# Autodesk Inventor assembly: Kolo+Opona
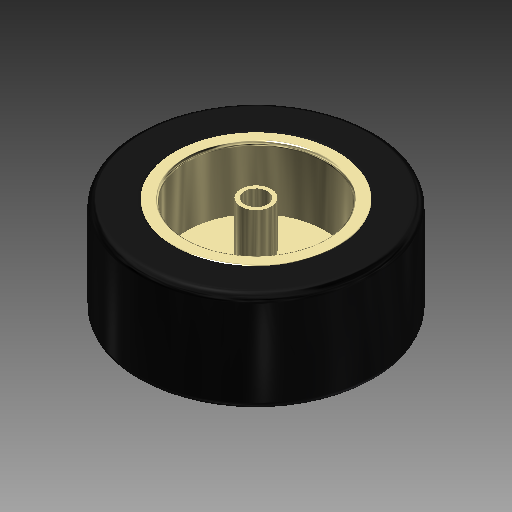
[picture p0: Inventor's stored thumbnail of the model, 512x512]
Saved by Autodesk Inventor 2017 (Build 210142000, 142)
## iProperties
Created: 2016-11-09
Part Number: Kolo+Opona
Document SubType Name: Assembly
Designer: Shichi
Author: Shichi
## Documents named in this file (3)
- C:\Users\Shichi\Desktop\TooStronk\Kolo+Opona.iam
- C:\Users\Shichi\Desktop\TooStronk\Opona.ipt
- C:\Users\Shichi\Desktop\TooStronk\Kolo.ipt
## Components (2 placed, 2 different names)
1. Opona:1 — Insert:1
2. Kolo:1 — Insert:1
## Relationships (1: Insert 1)
- Insert:1: Opona:1 ↔ Kolo:1
